# Autodesk Inventor assembly: Worm
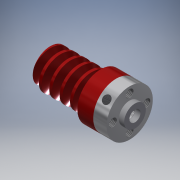
[picture p0: Inventor's stored thumbnail of the model, 180x180]
Saved by Autodesk Inventor 2019.1 (Build 231200000, 200)
## iProperties
Created: 2018-11-21
Part Number: Worm
Material: Generisch
Document SubType Name: Assembly
Designer: JochenAlt
Author: JochenAlt
## Documents named in this file (4)
- D:\Projects\Ondine\CAD\Leg\Worm.iam
- D:\Projects\Ondine\CAD\Leg\Schnecke\Schnecke1.ipt
- D:\Projects\Ondine\CAD\Leg\WormBushing.ipt
- D:\Projects\Ondine\CAD\Mounting Hub 3mm.ipt
## Components (3 placed, 3 different names)
1. Schnecke:1 — Passend:5, Passend:6, Passend:7
2. WormBushing:1 — Passend:3
3. Mounting Hub:1 — Passend:3, Passend:5, Passend:6, Passend:7
## Relationships (4: Mate 4)
- Passend:3 [Mate]: WormBushing:1 ↔ Mounting Hub:1
- Passend:5 [Mate]: Schnecke:1 ↔ Mounting Hub:1
- Passend:6 [Mate]: Schnecke:1 ↔ Mounting Hub:1
- Passend:7 [Mate]: Schnecke:1 ↔ Mounting Hub:1
